# Autodesk Inventor assembly: Robot
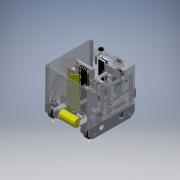
[picture p0: Inventor's stored thumbnail of the model, 180x180]
Saved by Autodesk Inventor 2017 (Build 210142000, 142)
## iProperties
Created: 2016-10-08
Part Number: Robot
Document SubType Name: Assembly
Designer: RoboticsUser
Author: RoboticsUser
## Documents named in this file (38)
- C:\Robotics\CAD\2016-17_CAD\Robot - CAD.iam
- C:\Robotics\CAD\2016-17_CAD\WheelAssemblyWFrame.iam
- C:\Robotics\CAD\COTSParts\Bosch Extrusion\Bosch 20x20 9 in.ipt
- C:\Robotics\CAD\COTSParts\Bosch Extrusion\Gusset 20x20 w screws.ipt
- C:\Robotics\CAD\COTSParts\Bosch Extrusion\Bosch 20x20 9 in - Copy.ipt
- C:\Robotics\CAD\COTSParts\Bosch Extrusion\Rexroth-6mmT-Nutm4.ipt
- C:\Robotics\CAD\COTSParts\Bosch Extrusion\Rexroth-GussetwFastenersm4x8.ipt
- C:\Robotics\CAD\COTSParts\Bosch Extrusion\Bosch 20x20 8.937in.ipt
- C:\Robotics\CAD\2016-17_CAD\ParticleLauncher2.0.iam
- C:\Robotics\CAD\2016-17_CAD\BBP.iam
- C:\Robotics\CAD\2016-17_CAD\ElectronicsPlate2.ipt
- C:\Robotics\CAD\2016-17_CAD\Deflecter.ipt
- C:\Robotics\CAD\COTSParts\Actobotics\585 parts\585424.ipt
- C:\Robotics\CAD\2016-17_CAD\14inLift - Copy.iam
- C:\Robotics\CAD\COTSParts\Bosch Extrusion\Bosch 20x20 4 14in.ipt
- C:\Robotics\CAD\2016-17_CAD\Backstop.iam
- C:\Robotics\CAD\COTSParts\Bosch Extrusion\Bosch 20x20 9 in actual2.ipt
- C:\Robotics\CAD\2016-17_CAD\CollectorPrototype.iam
- C:\Robotics\CAD\COTSParts\Actobotics\585 parts\585494.ipt
- C:\Robotics\CAD\COTSParts\Motors\Andymark 2964  NeveRest 40 Motor.ipt
- C:\Robotics\CAD\COTSParts\Actobotics\555 parts\555116.ipt
- C:\Robotics\CAD\2016-17_CAD\Motorstandoff1a1.2.ipt
- C:\Robotics\CAD\COTSParts\Actobotics\615 parts\615102.ipt
- C:\Robotics\CAD\2016-17_CAD\ModuleAssembly.iam
- C:\Robotics\CAD\COTSParts\ModernRobotics\MRI45-2203_Motor_Controller.ipt
- C:\Robotics\CAD\2016-17_CAD\Phone.ipt
- C:\Robotics\CAD\COTSParts\ModernRobotics\MRI45-2200_Power_Distribution_Module.ipt
- C:\Robotics\CAD\COTSParts\ModernRobotics\45-2018_Color.ipt
- C:\Robotics\CAD\COTSParts\Actobotics\am-3102NeveRest20 (1).ipt
- C:\Robotics\CAD\2016-17_CAD\CapLiftHolder.ipt
- C:\Robotics\CAD\2016-17_CAD\Lift.iam
- C:\Robotics\CAD\2016-17_CAD\LiftPully.ipt
- C:\Robotics\CAD\2016-17_CAD\LeftSidePlate.ipt
- C:\Robotics\CAD\COTSParts\Bosch Extrusion\Bosch 20x20 13 in - Real.ipt
- C:\Robotics\CAD\2016-17_CAD\HingeMK3.iam
- C:\Robotics\CAD\2016-17_CAD\MarbleTemplate.ipt
- C:\Robotics\CAD\2016-17_CAD\SidePlateFront.ipt
- C:\Robotics\CAD\2016-17_CAD\Boot.iam
## Components (69 placed, 37 different names)
1. WheelAssemblyWFrame:1 [sub-assembly] — Insert:4, Insert:5, Insert:6, Flush:29, Flush:37, Flush:114, Mate:181, Mate:226, Flush:134, Flush:138, Mate:269, Flush:157, Flush:158
2. WheelAssemblyWFrame:2 [sub-assembly] — Mate:8, Insert:1, Insert:2, Insert:3, Flush:30, Mate:57, Mate:58, Mate:77, Mate:192, Mate:194, Flush:122, Flush:123, Mate:198, Flush:124, Mate:201, Flush:125, Mate:203, Flush:126, Mate:260, Flush:148, Mate:261, Mate:271, Flush:161, Flush:162
3. Bosch 20x20 9 in:1 — Flush:37, Mate:56, Mate:58, Mate:77, Mate:227, Mate:230, Flush:136, Mate:232, Flush:138, Mate:252
4. Gusset 20x20 w screws:3 — Mate:8
5. Bosch 20x20 9 in - Copy:1 — Mate:33, Flush:25, Flush:30, Mate:175, Mate:183, Flush:115, Mate:244, Flush:143
6. Rexroth-6mmT-Nutm4:1 — Insert:1
7. Rexroth-6mmT-Nutm4:2 — Insert:3, Mate:33, Flush:25
8. Rexroth-6mmT-Nutm4:3 — Insert:2
9. Bosch 20x20 9 in - Copy:2 — Mate:15, Flush:11, Flush:29, Flush:116
10. Rexroth-6mmT-Nutm4:4 — Insert:4
11. Rexroth-6mmT-Nutm4:5 — Insert:5
12. Rexroth-6mmT-Nutm4:6 — Insert:6, Mate:15, Flush:11
13. Rexroth-GussetwFastenersm4x8:4 — Mate:56, Mate:57
14. Bosch 20x20 8.937in:4 — Mate:93, Flush:62, Flush:92, Flush:103, Flush:104, Mate:160
15. ParticleLauncher2.0:1 [sub-assembly] — Flush:103, Flush:104, Mate:160, Mate:163, Mate:164, Mate:165, Mate:166, Mate:168, Mate:169, Mate:170, Mate:171, Mate:174, Flush:113, Flush:114, Mate:181, Mate:206, Flush:127, Mate:208, Flush:128, Mate:209, Flush:141
16. Gusset 20x20 w screws:18 — Mate:93, Flush:62, Flush:92
17. BBP:1 [sub-assembly] — Mate:206, Flush:127, Flush:141, Flush:142
18. ElectronicsPlate2:1 — Mate:175, Mate:214
19. Deflecter:2 — Mate:174, Mate:177, Flush:112, Mate:179
20. 585424:2 — Insert:7, Insert:8, Flush:112, Mate:179, Flush:113
21. Rexroth-6mmT-Nutm4:7 — Mate:165, Mate:166, Insert:9
22. Rexroth-6mmT-Nutm4:8 — Mate:163, Mate:164, Insert:10
23. Rexroth-6mmT-Nutm4:10 — Mate:168, Mate:169, Insert:8
24. Rexroth-6mmT-Nutm4:11 — Mate:170, Mate:171, Insert:7
25. 585424:3 — Insert:9, Insert:10, Mate:177
26. 14inLift - Copy:1 [sub-assembly] — Mate:183, Flush:115, Flush:116, Mate:184, Flush:117, Mate:187, Mate:188, Flush:118, Mate:193, Flush:119, Flush:120, Flush:121, Mate:195, Mate:196, Mate:197, Insert:18, Mate:199, Mate:214, Tangent:3, Tangent:4
27. Bosch 20x20 4 14in:1 — Mate:184, Flush:117, Mate:185
28. Backstop:1 [sub-assembly] — Mate:185, Mate:190, Mate:191
29. Bosch 20x20 4 14in:2 — Mate:188, Flush:118, Mate:191, Flush:121
30. Bosch 20x20 4 14in:3 — Mate:187, Mate:190, Flush:120, Mate:267
31. Bosch 20x20 9 in actual2:1 — Mate:192, Mate:193, Flush:119
32. CollectorPrototype:1 [sub-assembly] — Mate:194, Flush:122, Flush:123
33. 585494:1 — Insert:11, Insert:12, Insert:13, Insert:14
34. Andymark 2964  NeveRest 40 Motor:1 — Insert:15, Insert:19
35. 555116:1 — Insert:15, Insert:16, Insert:17
36. Motorstandoff1a1.2:1 — Insert:12, Insert:17
37. Motorstandoff1a1.2:2 — Insert:11, Insert:16
38. Rexroth-6mmT-Nutm4:12 — Insert:13, Mate:195, Mate:196
39. Rexroth-6mmT-Nutm4:13 — Insert:14, Mate:197
40. 615102:1 — Insert:18
41. 615102:2 — Insert:19
42. ModuleAssembly:1 [sub-assembly] — Mate:198, Mate:199, Flush:124, Mate:200, Mate:202, Mate:204, Mate:205, Mate:210, Flush:129, Flush:130, Mate:211, Mate:212, Tangent:5
43. Gusset 20x20 w screws:23 — Mate:200, Mate:201, Flush:125
44. Gusset 20x20 w screws:24 — Mate:202, Mate:203, Flush:126
45. MRI45-2203_Motor_Controller:2 — Mate:204, Mate:205
46. Phone:1 — Mate:208, Flush:128, Mate:209
47. MRI45-2200_Power_Distribution_Module:1 — Mate:210, Flush:129, Flush:130
48. MRI45-2203_Motor_Controller:3 — Mate:211, Mate:212
49. 45-2018_Color:1 — Flush:142, Mate:243, Mate:247, Flush:251
50. 45-2018_Color:2 — Mate:243, Mate:248, Flush:252
51. am-3102NeveRest20 (1):1 — Insert:20
52. 555116:2 — Insert:20, Flush:145, Mate:265
53. Rexroth-GussetwFastenersm4x8:5 — Mate:226, Flush:134, Mate:227
54. CapLiftHolder:1 — Mate:232, Flush:146
55. CapLiftHolder:2 — Mate:230, Flush:136, Mate:253
56. CapLiftHolder:3 — Mate:251, Mate:254
57. Bosch 20x20 9 in:2 — Mate:244, Flush:143, Mate:247, Mate:248, Flush:252, Flush:251, Mate:251, Flush:144, Mate:264
58. Lift:1 [sub-assembly] — Mate:252, Flush:144, Mate:253, Mate:254, Flush:145, Flush:146, Mate:255, Tangent:1, Tangent:2, Mate:256, Mate:264, Mate:265, Mate:266, Flush:153, Flush:154
59. LiftPully:1 — Mate:255, Tangent:1, Tangent:2, Mate:257
60. CapLiftHolder:4 — Mate:256, Mate:257
61. LeftSidePlate:1 — Mate:260, Flush:148, Mate:261, Mate:262, Flush:149, Flush:150, Mate:263, Flush:151, Flush:152
62. Bosch 20x20 13 in - Real:1 — Mate:262, Flush:149, Flush:150, Mate:268, Flush:155, Flush:156
63. Bosch 20x20 13 in - Real:2 — Mate:263, Flush:151, Flush:152
64. HingeMK3:1 [sub-assembly] — Mate:266, Flush:153, Flush:154
65. MarbleTemplate:1 — Mate:267, Tangent:3, Tangent:4, Tangent:5
66. SidePlateFront:1 — Mate:268, Flush:155, Flush:156
67. Bosch 20x20 13 in - Real:3 — Mate:269, Flush:157, Flush:158, Mate:270, Flush:159, Flush:160
68. LeftSidePlate:2 — Mate:270, Flush:159, Flush:160
69. Boot:1 [sub-assembly] — Mate:271, Flush:161, Flush:162
## Relationships (156: Mate 77, Flush 54, Insert 20, Tangent 5)
- Mate:8: WheelAssemblyWFrame:2 ↔ Gusset 20x20 w screws:3
- Insert:1: WheelAssemblyWFrame:2 ↔ Rexroth-6mmT-Nutm4:1
- Insert:2: WheelAssemblyWFrame:2 ↔ Rexroth-6mmT-Nutm4:3
- Insert:3: WheelAssemblyWFrame:2 ↔ Rexroth-6mmT-Nutm4:2
- Insert:4: WheelAssemblyWFrame:1 ↔ Rexroth-6mmT-Nutm4:4
- Insert:5: WheelAssemblyWFrame:1 ↔ Rexroth-6mmT-Nutm4:5
- Insert:6: WheelAssemblyWFrame:1 ↔ Rexroth-6mmT-Nutm4:6
- Mate:15: Bosch 20x20 9 in - Copy:2 ↔ Rexroth-6mmT-Nutm4:6
- Flush:11 (64.77 mm): Bosch 20x20 9 in - Copy:2 ↔ Rexroth-6mmT-Nutm4:6
- Mate:33: Bosch 20x20 9 in - Copy:1 ↔ Rexroth-6mmT-Nutm4:2
- Flush:25 (64.77 mm): Bosch 20x20 9 in - Copy:1 ↔ Rexroth-6mmT-Nutm4:2
- Flush:29 (1.6256 mm): WheelAssemblyWFrame:1 ↔ Bosch 20x20 9 in - Copy:2
- Flush:30 (1.6256 mm): WheelAssemblyWFrame:2 ↔ Bosch 20x20 9 in - Copy:1
- Flush:37: WheelAssemblyWFrame:1 ↔ Bosch 20x20 9 in:1
- Mate:56: Bosch 20x20 9 in:1 ↔ Rexroth-GussetwFastenersm4x8:4
- Mate:57: WheelAssemblyWFrame:2 ↔ Rexroth-GussetwFastenersm4x8:4
- Mate:58: WheelAssemblyWFrame:2 ↔ Bosch 20x20 9 in:1
- Mate:77: WheelAssemblyWFrame:2 ↔ Bosch 20x20 9 in:1
- Mate:93: Bosch 20x20 8.937in:4 ↔ Gusset 20x20 w screws:18
- Flush:62: Bosch 20x20 8.937in:4 ↔ Gusset 20x20 w screws:18
- Flush:92: Bosch 20x20 8.937in:4 ↔ Gusset 20x20 w screws:18
- Flush:103: Bosch 20x20 8.937in:4 ↔ ParticleLauncher2.0:1
- Flush:104: Bosch 20x20 8.937in:4 ↔ ParticleLauncher2.0:1
- Mate:160: Bosch 20x20 8.937in:4 ↔ ParticleLauncher2.0:1
- Mate:163: ParticleLauncher2.0:1 ↔ Rexroth-6mmT-Nutm4:8
- Mate:164: ParticleLauncher2.0:1 ↔ Rexroth-6mmT-Nutm4:8
- Mate:165: ParticleLauncher2.0:1 ↔ Rexroth-6mmT-Nutm4:7
- Mate:166: ParticleLauncher2.0:1 ↔ Rexroth-6mmT-Nutm4:7
- Mate:168: ParticleLauncher2.0:1 ↔ Rexroth-6mmT-Nutm4:10
- Mate:169: ParticleLauncher2.0:1 ↔ Rexroth-6mmT-Nutm4:10
- Mate:170: ParticleLauncher2.0:1 ↔ Rexroth-6mmT-Nutm4:11
- Mate:171: ParticleLauncher2.0:1 ↔ Rexroth-6mmT-Nutm4:11
- Mate:174: ParticleLauncher2.0:1 ↔ Deflecter:2
- Mate:175: Bosch 20x20 9 in - Copy:1 ↔ ElectronicsPlate2:1
- Insert:7: 585424:2 ↔ Rexroth-6mmT-Nutm4:11
- Insert:8: 585424:2 ↔ Rexroth-6mmT-Nutm4:10
- Insert:9: Rexroth-6mmT-Nutm4:7 ↔ 585424:3
- Insert:10: Rexroth-6mmT-Nutm4:8 ↔ 585424:3
- Mate:177: Deflecter:2 ↔ 585424:3
- Flush:112 (2.54 mm): Deflecter:2 ↔ 585424:2
- Mate:179: Deflecter:2 ↔ 585424:2
- Flush:113 (-88.9 mm): ParticleLauncher2.0:1 ↔ 585424:2
- Flush:114: WheelAssemblyWFrame:1 ↔ ParticleLauncher2.0:1
- Mate:181: WheelAssemblyWFrame:1 ↔ ParticleLauncher2.0:1
- Mate:183: Bosch 20x20 9 in - Copy:1 ↔ 14inLift - Copy:1
- Flush:115: Bosch 20x20 9 in - Copy:1 ↔ 14inLift - Copy:1
- Flush:116 (114.3 mm): Bosch 20x20 9 in - Copy:2 ↔ 14inLift - Copy:1
- Mate:184: 14inLift - Copy:1 ↔ Bosch 20x20 4 14in:1
- Flush:117: 14inLift - Copy:1 ↔ Bosch 20x20 4 14in:1
- Mate:185: Bosch 20x20 4 14in:1 ↔ Backstop:1
- Mate:187: 14inLift - Copy:1 ↔ Bosch 20x20 4 14in:3
- Mate:188: 14inLift - Copy:1 ↔ Bosch 20x20 4 14in:2
- Flush:118 (76.2 mm): 14inLift - Copy:1 ↔ Bosch 20x20 4 14in:2
- Mate:190: Backstop:1 ↔ Bosch 20x20 4 14in:3
- Mate:191: Backstop:1 ↔ Bosch 20x20 4 14in:2
- Mate:192: WheelAssemblyWFrame:2 ↔ Bosch 20x20 9 in actual2:1
- Mate:193: 14inLift - Copy:1 ↔ Bosch 20x20 9 in actual2:1
- Flush:119: 14inLift - Copy:1 ↔ Bosch 20x20 9 in actual2:1
- Flush:120: 14inLift - Copy:1 ↔ Bosch 20x20 4 14in:3
- Flush:121: 14inLift - Copy:1 ↔ Bosch 20x20 4 14in:2
- Mate:194: WheelAssemblyWFrame:2 ↔ CollectorPrototype:1
- Flush:122: WheelAssemblyWFrame:2 ↔ CollectorPrototype:1
- Flush:123 (25.4 mm): WheelAssemblyWFrame:2 ↔ CollectorPrototype:1
- Insert:11: 585494:1 ↔ Motorstandoff1a1.2:2
- Insert:12: 585494:1 ↔ Motorstandoff1a1.2:1
- Insert:13: 585494:1 ↔ Rexroth-6mmT-Nutm4:12
- Insert:14: 585494:1 ↔ Rexroth-6mmT-Nutm4:13
- Insert:15: Andymark 2964  NeveRest 40 Motor:1 ↔ 555116:1
- Insert:16: 555116:1 ↔ Motorstandoff1a1.2:2
- Insert:17: 555116:1 ↔ Motorstandoff1a1.2:1
- Mate:195: 14inLift - Copy:1 ↔ Rexroth-6mmT-Nutm4:12
- Mate:196: 14inLift - Copy:1 ↔ Rexroth-6mmT-Nutm4:12
- Mate:197: 14inLift - Copy:1 ↔ Rexroth-6mmT-Nutm4:13
- Insert:18 (7.62 mm): 14inLift - Copy:1 ↔ 615102:1
- Insert:19 (2.54 mm): Andymark 2964  NeveRest 40 Motor:1 ↔ 615102:2
- Mate:198: WheelAssemblyWFrame:2 ↔ ModuleAssembly:1
- Mate:199: 14inLift - Copy:1 ↔ ModuleAssembly:1
- Flush:124: WheelAssemblyWFrame:2 ↔ ModuleAssembly:1
- Mate:200: ModuleAssembly:1 ↔ Gusset 20x20 w screws:23
- Mate:201: WheelAssemblyWFrame:2 ↔ Gusset 20x20 w screws:23
- Flush:125: WheelAssemblyWFrame:2 ↔ Gusset 20x20 w screws:23
- Mate:202: ModuleAssembly:1 ↔ Gusset 20x20 w screws:24
- Mate:203: WheelAssemblyWFrame:2 ↔ Gusset 20x20 w screws:24
- Flush:126: WheelAssemblyWFrame:2 ↔ Gusset 20x20 w screws:24
- Mate:204: ModuleAssembly:1 ↔ MRI45-2203_Motor_Controller:2
- Mate:205: ModuleAssembly:1 ↔ MRI45-2203_Motor_Controller:2
- Mate:206: ParticleLauncher2.0:1 ↔ BBP:1
- Flush:127: ParticleLauncher2.0:1 ↔ BBP:1
- Mate:208: ParticleLauncher2.0:1 ↔ Phone:1
- Flush:128: ParticleLauncher2.0:1 ↔ Phone:1
- Mate:209: ParticleLauncher2.0:1 ↔ Phone:1
- Mate:210: ModuleAssembly:1 ↔ MRI45-2200_Power_Distribution_Module:1
- Flush:129: ModuleAssembly:1 ↔ MRI45-2200_Power_Distribution_Module:1
- Flush:130 (63.5 mm): ModuleAssembly:1 ↔ MRI45-2200_Power_Distribution_Module:1
- Mate:211: ModuleAssembly:1 ↔ MRI45-2203_Motor_Controller:3
- Mate:212: ModuleAssembly:1 ↔ MRI45-2203_Motor_Controller:3
- Mate:214: ElectronicsPlate2:1 ↔ 14inLift - Copy:1
- Insert:20: am-3102NeveRest20 (1):1 ↔ 555116:2
- Mate:226: WheelAssemblyWFrame:1 ↔ Rexroth-GussetwFastenersm4x8:5
- Flush:134: WheelAssemblyWFrame:1 ↔ Rexroth-GussetwFastenersm4x8:5
- Mate:227: Bosch 20x20 9 in:1 ↔ Rexroth-GussetwFastenersm4x8:5
- Mate:230: Bosch 20x20 9 in:1 ↔ CapLiftHolder:2
- Flush:136: Bosch 20x20 9 in:1 ↔ CapLiftHolder:2
- Mate:232: Bosch 20x20 9 in:1 ↔ CapLiftHolder:1
- Flush:138 (70.9422 mm): WheelAssemblyWFrame:1 ↔ Bosch 20x20 9 in:1
- Flush:141 (-50.8 mm): ParticleLauncher2.0:1 ↔ BBP:1
- Flush:142: BBP:1 ↔ 45-2018_Color:1
- Mate:243 (12.7 mm): 45-2018_Color:1 ↔ 45-2018_Color:2
- Mate:244: Bosch 20x20 9 in - Copy:1 ↔ Bosch 20x20 9 in:2
- Flush:143: Bosch 20x20 9 in - Copy:1 ↔ Bosch 20x20 9 in:2
- Mate:247: 45-2018_Color:1 ↔ Bosch 20x20 9 in:2
- Mate:248: 45-2018_Color:2 ↔ Bosch 20x20 9 in:2
- Flush:252: 45-2018_Color:2 ↔ Bosch 20x20 9 in:2
- Flush:251: 45-2018_Color:1 ↔ Bosch 20x20 9 in:2
- Mate:251: CapLiftHolder:3 ↔ Bosch 20x20 9 in:2
- Mate:252: Bosch 20x20 9 in:1 ↔ Lift:1
- Flush:144: Bosch 20x20 9 in:2 ↔ Lift:1
- Mate:253: CapLiftHolder:2 ↔ Lift:1
- Mate:254: CapLiftHolder:3 ↔ Lift:1
- Flush:145 (177.8 mm): 555116:2 ↔ Lift:1
- Flush:146: CapLiftHolder:1 ↔ Lift:1
- Mate:255: Lift:1 ↔ LiftPully:1
- Tangent:1: Lift:1 ↔ LiftPully:1
- Tangent:2 (-152.4 mm): Lift:1 ↔ LiftPully:1
- Mate:256: Lift:1 ↔ CapLiftHolder:4
- Mate:257: LiftPully:1 ↔ CapLiftHolder:4
- Mate:260: WheelAssemblyWFrame:2 ↔ LeftSidePlate:1
- Flush:148: WheelAssemblyWFrame:2 ↔ LeftSidePlate:1
- Mate:261: WheelAssemblyWFrame:2 ↔ LeftSidePlate:1
- Mate:262: LeftSidePlate:1 ↔ Bosch 20x20 13 in - Real:1
- Flush:149: LeftSidePlate:1 ↔ Bosch 20x20 13 in - Real:1
- Flush:150: LeftSidePlate:1 ↔ Bosch 20x20 13 in - Real:1
- Mate:263: LeftSidePlate:1 ↔ Bosch 20x20 13 in - Real:2
- Flush:151: LeftSidePlate:1 ↔ Bosch 20x20 13 in - Real:2
- Flush:152: LeftSidePlate:1 ↔ Bosch 20x20 13 in - Real:2
- Mate:264: Bosch 20x20 9 in:2 ↔ Lift:1
- Mate:265: 555116:2 ↔ Lift:1
- Mate:266: Lift:1 ↔ HingeMK3:1
- Flush:153: Lift:1 ↔ HingeMK3:1
- Flush:154 (13.081 mm): Lift:1 ↔ HingeMK3:1
- Mate:267: Bosch 20x20 4 14in:3 ↔ MarbleTemplate:1
- Mate:268: Bosch 20x20 13 in - Real:1 ↔ SidePlateFront:1
- Flush:155: Bosch 20x20 13 in - Real:1 ↔ SidePlateFront:1
- Flush:156: Bosch 20x20 13 in - Real:1 ↔ SidePlateFront:1
- Mate:269: WheelAssemblyWFrame:1 ↔ Bosch 20x20 13 in - Real:3
- Flush:157: WheelAssemblyWFrame:1 ↔ Bosch 20x20 13 in - Real:3
- Flush:158: WheelAssemblyWFrame:1 ↔ Bosch 20x20 13 in - Real:3
- Mate:270: Bosch 20x20 13 in - Real:3 ↔ LeftSidePlate:2
- Flush:159: Bosch 20x20 13 in - Real:3 ↔ LeftSidePlate:2
- Flush:160: Bosch 20x20 13 in - Real:3 ↔ LeftSidePlate:2
- Tangent:3: 14inLift - Copy:1 ↔ MarbleTemplate:1
- Tangent:4: 14inLift - Copy:1 ↔ MarbleTemplate:1
- Tangent:5: ModuleAssembly:1 ↔ MarbleTemplate:1
- Mate:271: WheelAssemblyWFrame:2 ↔ Boot:1
- Flush:161: WheelAssemblyWFrame:2 ↔ Boot:1
- Flush:162 (27.0256 mm): WheelAssemblyWFrame:2 ↔ Boot:1
